# Autodesk Inventor assembly: ラマン分光系
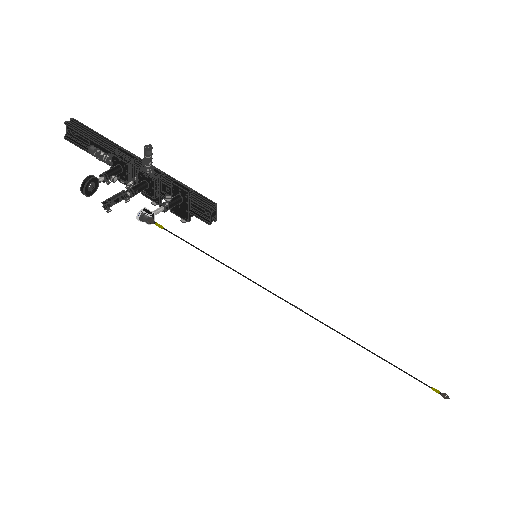
[picture p0: Inventor's stored thumbnail of the model, 512x512]
Saved by Autodesk Inventor 2026.2 (Build 302298000, 298)
## iProperties
Created: 2025-07-11
Part Number: ラマン分光系
Document SubType Name: Assembly
Designer: jin20
Author: jin20
## Documents named in this file (8)
- D:\repos\PIHTI\SpectroscopySystem_Hayashi\ラマン分光系.iam
- D:\repos\PIHTI\SpectroscopySystem_Hayashi\Stage\光学レール.ipt
- D:\repos\PIHTI\SpectroscopySystem_Hayashi\Stage\レールキャリア.ipt
- D:\repos\PIHTI\SpectroscopySystem_Hayashi\Optics\レンズ_f100.iam
- D:\repos\PIHTI\SpectroscopySystem_Hayashi\Stage\手動ステージ\手動ステージ.iam
- D:\repos\PIHTI\SpectroscopySystem_Hayashi\Optics\ダイクロイックミラー.iam
- D:\repos\PIHTI\SpectroscopySystem_Hayashi\Optics\コリメータ_エッジフィルター.iam
- D:\repos\PIHTI\SpectroscopySystem_Hayashi\Optics\光ファイバー.ipt
## Components (10 placed, 7 different names)
1. 光学レール:1 — スライダ:1, スライダ:2, スライダ:3
2. レールキャリア:1 — スライダ:2, 挿入:6, 挿入:7, 挿入:8, 挿入:9, 挿入:10
3. レールキャリア:2 — スライダ:3, 挿入:1, 挿入:2, 挿入:3, 挿入:4
4. レールキャリア:3 — スライダ:1, 挿入:11
5. レンズ_f100:1 [sub-assembly] — 挿入:5
6. 手動ステージ:1 [sub-assembly] — 挿入:1, 挿入:2, 挿入:3, 挿入:4, 挿入:5
7. 手動ステージ:2 [sub-assembly] — 挿入:6, 挿入:7, 挿入:8, 挿入:9, 挿入:10, 回転:1
8. ダイクロイックミラー:1 [sub-assembly] — 回転:1
9. コリメータ_エッジフィルター:1 [sub-assembly] — 挿入:11, 挿入:12
10. 光ファイバー:1 — 挿入:12
## Relationships (16: Insert 12, TranslationJoint 3, RevoluteJoint 1)
- スライダ:1 [TranslationJoint]: 光学レール:1 ↔ レールキャリア:3
- スライダ:2 [TranslationJoint]: 光学レール:1 ↔ レールキャリア:1
- スライダ:3 [TranslationJoint]: 光学レール:1 ↔ レールキャリア:2
- 挿入:1 [Insert]: レールキャリア:2 ↔ 手動ステージ:1
- 挿入:2 [Insert]: レールキャリア:2 ↔ 手動ステージ:1
- 挿入:3 [Insert]: レールキャリア:2 ↔ 手動ステージ:1
- 挿入:4 [Insert]: レールキャリア:2 ↔ 手動ステージ:1
- 挿入:5 [Insert]: レンズ_f100:1 ↔ 手動ステージ:1
- 挿入:6 [Insert]: レールキャリア:1 ↔ 手動ステージ:2
- 挿入:7 [Insert]: レールキャリア:1 ↔ 手動ステージ:2
- 挿入:8 [Insert]: レールキャリア:1 ↔ 手動ステージ:2
- 挿入:9 [Insert]: レールキャリア:1 ↔ 手動ステージ:2
- 挿入:10 [Insert]: レールキャリア:1 ↔ 手動ステージ:2
- 回転:1 [RevoluteJoint]: 手動ステージ:2 ↔ ダイクロイックミラー:1
- 挿入:11 [Insert]: レールキャリア:3 ↔ コリメータ_エッジフィルター:1
- 挿入:12 [Insert]: コリメータ_エッジフィルター:1 ↔ 光ファイバー:1
